# Autodesk Inventor assembly: RT_ELE_002_ElectricalMainPlate
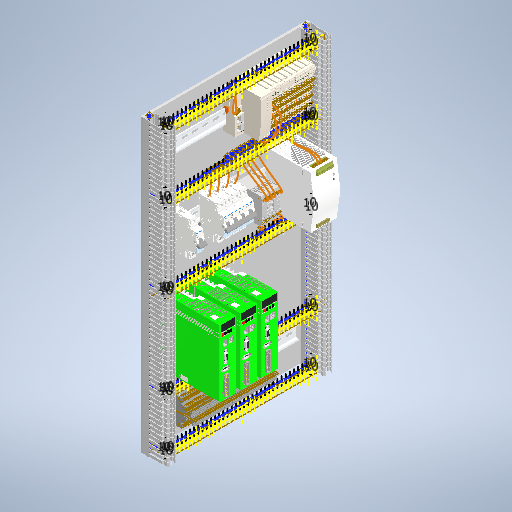
[picture p0: Inventor's stored thumbnail of the model, 512x512]
Saved by Autodesk Inventor 2025.3 (Build 293356000, 356)
## iProperties
Created: 2026-06-07
Part Number: RT_ELE_002_ElectricalMainPlate
Document SubType Name: Assembly
Designer: louis
Author: louis
## Documents named in this file (14)
- C:\Users\louis\OneDrive\Desktop\R_Trident\02_CAD\04_Subassemblies\RT_ELE_001_ElectricalMainPlate_V0.2.iam
- C:\Users\louis\OneDrive\Desktop\R_Trident\02_CAD\01_Standard_Parts\04_ELE_Electrical_Automation\A6-400EC\A6-400EC.iam
- C:\Users\louis\OneDrive\Desktop\R_Trident\02_CAD\01_Standard_Parts\04_ELE_Electrical_Automation\DIN RAIL STEEL.ipt
- C:\Users\louis\OneDrive\Desktop\R_Trident\02_CAD\03_Parts_Custom\RT_ELE_MC_017_MainBackPlate.ipt
- C:\Users\louis\OneDrive\Desktop\R_Trident\02_CAD\01_Standard_Parts\04_ELE_Electrical_Automation\Cable channel 60x25\Cable channel 60x25x700.ipt
- C:\Users\louis\OneDrive\Desktop\R_Trident\02_CAD\01_Standard_Parts\04_ELE_Electrical_Automation\Cable channel 60x25\Cable channel 60x25x350.ipt
- C:\Users\louis\OneDrive\Desktop\R_Trident\02_CAD\01_Standard_Parts\04_ELE_Electrical_Automation\NFN 102\NCN013.ipt
- C:\Users\louis\OneDrive\Desktop\R_Trident\02_CAD\01_Standard_Parts\04_ELE_Electrical_Automation\NFN 102\NCN006.ipt
- C:\Users\louis\OneDrive\Desktop\R_Trident\02_CAD\01_Standard_Parts\04_ELE_Electrical_Automation\dilm7-10_24vdc_.ipt
- C:\Users\louis\OneDrive\Desktop\R_Trident\02_CAD\01_Standard_Parts\04_ELE_Electrical_Automation\WagoIO\Wago_IO_Module.iam
- C:\Users\louis\OneDrive\Desktop\R_Trident\02_CAD\01_Standard_Parts\04_ELE_Electrical_Automation\WagoIO\IO.iam
- C:\Users\louis\OneDrive\Desktop\R_Trident\02_CAD\01_Standard_Parts\04_ELE_Electrical_Automation\wdr_240_24\WDR-240-24.iam
- C:\Users\louis\OneDrive\Desktop\R_Trident\02_CAD\04_Subassemblies\RT_ELE_001_ElectricalMainPlate_V0.2\AIP\Cable and Harness\RT_ELE_001_ElectricalMainPlate_V0.2.Mains_230V.iam
- C:\Users\louis\OneDrive\Desktop\R_Trident\02_CAD\04_Subassemblies\RT_ELE_001_ElectricalMainPlate_V0.2\AIP\Cable and Harness\RT_ELE_001_ElectricalMainPlate_V0.2.LowVoltage_~24V.iam
## Components (25 placed, 13 different names)
1. A6-400EC:1 [sub-assembly] — Mate:26, Mate:27
2. A6-400EC:2 [sub-assembly] — Mate:24, Mate:25
3. A6-400EC:3 [sub-assembly] — Mate:22, Mate:23
4. RT_ELE_MC_017_MainBackPlate:1 — Mate:1, Mate:21, Mate:20, Flush:1, Mate:4, Mate:5, Flush:2, Mate:6, Flush:3, Flush:4, Mate:8, Mate:10, Flush:5, Mate:11, Mate:14, Mate:17, Mate:22, Mate:23, Mate:24, Mate:25, Mate:26, Mate:27, Mate:28, Mate:31, Mate:33
5. Cable channel 60x25x700:1 — Flush:1, Mate:4, Mate:5
6. Cable channel 60x25x700:2 — Flush:2, Mate:6, Flush:3, Mate:7, Mate:9, Mate:12, Mate:15, Mate:18, Mate:30, Mate:32, Mate:34
7. Cable channel 60x25x350:1 — Mate:17, Mate:18, Mate:19, Symmetry:3
8. Cable channel 60x25x350:2 — Mate:11, Mate:12, Mate:13, Mate:16, Symmetry:1, Symmetry:2
9. Cable channel 60x25x350:3 — Mate:14, Mate:15, Mate:16, Mate:19, Symmetry:2
10. Cable channel 60x25x350:4 — Mate:9, Mate:10, Flush:5, Mate:13, Symmetry:1
11. Cable channel 60x25x350:5 — Flush:4, Mate:7, Mate:8, Symmetry:3
12. DIN RAIL STEEL:1 — Mate:28, Mate:29, Mate:30, Flush:9, Mate:56, Flush:10
13. DIN RAIL STEEL:2 — Mate:31, Mate:32, Flush:6, Mate:54, Mate:53, Mate:55
14. DIN RAIL STEEL:3 — Mate:33, Mate:34, Mate:35, Mate:40, Mate:42, Mate:44, Mate:46, Mate:48, Mate:52, Mate:57, Mate:58, Flush:11
15. NCN013:1 — Mate:41, Mate:42
16. NCN006:1 — Mate:43, Mate:44, Mate:50, Mate:51
17. NCN006:2 — Mate:47, Mate:48, Mate:49, Mate:50
18. NCN006:3 — Mate:45, Mate:46, Mate:51
19. NCN006:4 — Mate:39, Mate:40, Mate:49
20. dilm7-10_24vdc_:1 — Flush:8, Mate:52
21. Wago_IO_Module:1 [sub-assembly] — Mate:54, Mate:53, Mate:55
22. IO:1 [sub-assembly] — Flush:9, Mate:56, Flush:10
23. WDR-240-24:1 [sub-assembly] — Mate:57, Mate:58, Flush:11
24. RT_ELE_001_ElectricalMainPlate_V0.2.Mains_230V [sub-assembly]
25. RT_ELE_001_ElectricalMainPlate_V0.2.LowVoltage_~24V [sub-assembly]
## Relationships (66: Mate 53, Flush 10, Symmetry 3)
- Mate:1: RT_ELE_MC_017_MainBackPlate:1
- Mate:21: RT_ELE_MC_017_MainBackPlate:1
- Mate:20: RT_ELE_MC_017_MainBackPlate:1
- Flush:1: RT_ELE_MC_017_MainBackPlate:1 ↔ Cable channel 60x25x700:1
- Mate:4: RT_ELE_MC_017_MainBackPlate:1 ↔ Cable channel 60x25x700:1
- Mate:5: RT_ELE_MC_017_MainBackPlate:1 ↔ Cable channel 60x25x700:1
- Flush:2: RT_ELE_MC_017_MainBackPlate:1 ↔ Cable channel 60x25x700:2
- Mate:6: RT_ELE_MC_017_MainBackPlate:1 ↔ Cable channel 60x25x700:2
- Flush:3: RT_ELE_MC_017_MainBackPlate:1 ↔ Cable channel 60x25x700:2
- Flush:4: RT_ELE_MC_017_MainBackPlate:1 ↔ Cable channel 60x25x350:5
- Mate:7: Cable channel 60x25x700:2 ↔ Cable channel 60x25x350:5
- Mate:8: RT_ELE_MC_017_MainBackPlate:1 ↔ Cable channel 60x25x350:5
- Mate:9: Cable channel 60x25x700:2 ↔ Cable channel 60x25x350:4
- Mate:10: RT_ELE_MC_017_MainBackPlate:1 ↔ Cable channel 60x25x350:4
- Flush:5: RT_ELE_MC_017_MainBackPlate:1 ↔ Cable channel 60x25x350:4
- Mate:11: RT_ELE_MC_017_MainBackPlate:1 ↔ Cable channel 60x25x350:2
- Mate:12: Cable channel 60x25x700:2 ↔ Cable channel 60x25x350:2
- Mate:13 (130 mm): Cable channel 60x25x350:2 ↔ Cable channel 60x25x350:4
- Mate:14: RT_ELE_MC_017_MainBackPlate:1 ↔ Cable channel 60x25x350:3
- Mate:15: Cable channel 60x25x700:2 ↔ Cable channel 60x25x350:3
- Mate:16 (165 mm): Cable channel 60x25x350:2 ↔ Cable channel 60x25x350:3
- Mate:17: RT_ELE_MC_017_MainBackPlate:1 ↔ Cable channel 60x25x350:1
- Mate:18: Cable channel 60x25x700:2 ↔ Cable channel 60x25x350:1
- Mate:19 (185 mm): Cable channel 60x25x350:1 ↔ Cable channel 60x25x350:3
- Mate:22: A6-400EC:3 ↔ RT_ELE_MC_017_MainBackPlate:1
- Mate:23: A6-400EC:3 ↔ RT_ELE_MC_017_MainBackPlate:1
- Mate:24: A6-400EC:2 ↔ RT_ELE_MC_017_MainBackPlate:1
- Mate:25: A6-400EC:2 ↔ RT_ELE_MC_017_MainBackPlate:1
- Mate:26: A6-400EC:1 ↔ RT_ELE_MC_017_MainBackPlate:1
- Mate:27: A6-400EC:1 ↔ RT_ELE_MC_017_MainBackPlate:1
- Mate:28: RT_ELE_MC_017_MainBackPlate:1 ↔ DIN RAIL STEEL:1
- Mate:29: DIN RAIL STEEL:1
- Mate:30 (10 mm): Cable channel 60x25x700:2 ↔ DIN RAIL STEEL:1
- Mate:31: RT_ELE_MC_017_MainBackPlate:1 ↔ DIN RAIL STEEL:2
- Mate:32 (10 mm): Cable channel 60x25x700:2 ↔ DIN RAIL STEEL:2
- Symmetry:1: Cable channel 60x25x350:2 ↔ Cable channel 60x25x350:4
- Flush:6: DIN RAIL STEEL:2
- Mate:33: RT_ELE_MC_017_MainBackPlate:1 ↔ DIN RAIL STEEL:3
- Mate:34 (10 mm): Cable channel 60x25x700:2 ↔ DIN RAIL STEEL:3
- Symmetry:2: Cable channel 60x25x350:2 ↔ Cable channel 60x25x350:3
- Mate:35: DIN RAIL STEEL:3
- Symmetry:3: Cable channel 60x25x350:1 ↔ Cable channel 60x25x350:5
- Mate:39: NCN006:4
- Mate:40: DIN RAIL STEEL:3 ↔ NCN006:4
- Mate:41: NCN013:1
- Mate:42: DIN RAIL STEEL:3 ↔ NCN013:1
- Mate:43: NCN006:1
- Mate:44: DIN RAIL STEEL:3 ↔ NCN006:1
- Mate:45: NCN006:3
- Mate:46: DIN RAIL STEEL:3 ↔ NCN006:3
- Mate:47: NCN006:2
- Mate:48: DIN RAIL STEEL:3 ↔ NCN006:2
- Mate:49: NCN006:2 ↔ NCN006:4
- Mate:50: NCN006:1 ↔ NCN006:2
- Mate:51: NCN006:1 ↔ NCN006:3
- Flush:8: dilm7-10_24vdc_:1
- Mate:52: DIN RAIL STEEL:3 ↔ dilm7-10_24vdc_:1
- Mate:54: DIN RAIL STEEL:2 ↔ Wago_IO_Module:1
- Mate:53: DIN RAIL STEEL:2 ↔ Wago_IO_Module:1
- Mate:55 (20 mm): DIN RAIL STEEL:2 ↔ Wago_IO_Module:1
- Flush:9: DIN RAIL STEEL:1 ↔ IO:1
- Mate:56: DIN RAIL STEEL:1 ↔ IO:1
- Flush:10 (20 mm): DIN RAIL STEEL:1 ↔ IO:1
- Mate:57: DIN RAIL STEEL:3 ↔ WDR-240-24:1
- Mate:58: DIN RAIL STEEL:3 ↔ WDR-240-24:1
- Flush:11 (20 mm): DIN RAIL STEEL:3 ↔ WDR-240-24:1
